# Autodesk Inventor assembly: ASY MSC 120 support
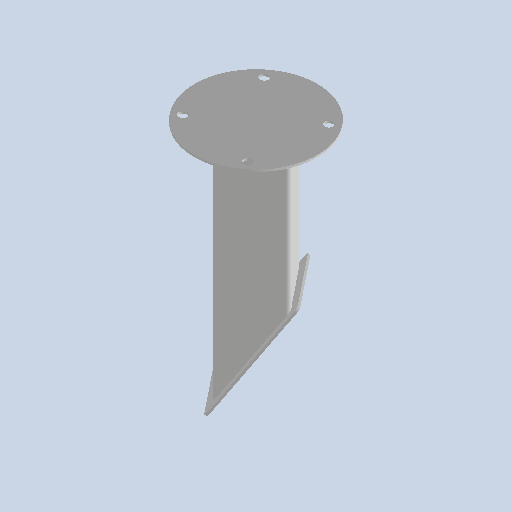
[picture p0: Inventor's stored thumbnail of the model, 512x512]
Saved by Autodesk Inventor 2025 (Build 290162010, 162A)
## iProperties
Created: 2024-08-15
Part Number: ASY MSC 120 support
Document SubType Name: Assembly
Designer: admin
Author: admin
## Documents named in this file (4)
- C:\Users\user\YandexDisk\домашниий пк\Inventor\Manturovo\Manturovo_Se-clar\ASY MSC 120 support.iam
- C:\Users\user\YandexDisk\домашниий пк\Inventor\Manturovo\Manturovo_Se-clar\MSC 125 base tube.ipt
- C:\Users\user\YandexDisk\домашниий пк\Inventor\Manturovo\Manturovo_Se-clar\MSC 126 flange base tube.ipt
- C:\Users\user\YandexDisk\домашниий пк\Inventor\Manturovo\Manturovo_Se-clar\MSC 128 flange base tube support.ipt
## Components (3 placed, 3 different names)
1. MSC 125 base tube:1
2. MSC 126 flange base tube:1
3. MSC 128 flange base tube support:1
## Relationships (2: WeldJoint 2)
- [WeldJoint]: MSC 125 base tube:1 ↔ MSC 126 flange base tube:1
- [WeldJoint]: MSC 125 base tube:1 ↔ MSC 128 flange base tube support:1
